# Autodesk Inventor assembly: Fender
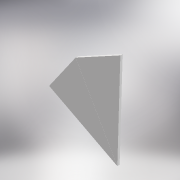
[picture p0: Inventor's stored thumbnail of the model, 180x180]
Saved by Autodesk Inventor 2020 (Build 240168000, 168)
## iProperties
Created: 2019-05-26
Part Number: Fender
Document SubType Name: Assembly
Designer: chitl
Author: chitl
## Documents named in this file (3)
- C:\Users\chitl\Desktop\OneWheel\Wheel Assembled\Fender\Fender.iam
- C:\Users\chitl\Desktop\OneWheel\Wheel Assembled\Fender\1.ipt
- C:\Users\chitl\Desktop\OneWheel\Wheel Assembled\Fender\2.ipt
## Components (2 placed, 2 different names)
1. 1:1 — Rigid:1
2. 2:1 — Rigid:1
## Relationships (1: WeldJoint 1)
- Rigid:1 [WeldJoint]: 1:1 ↔ 2:1
